# Autodesk Inventor assembly: board_box
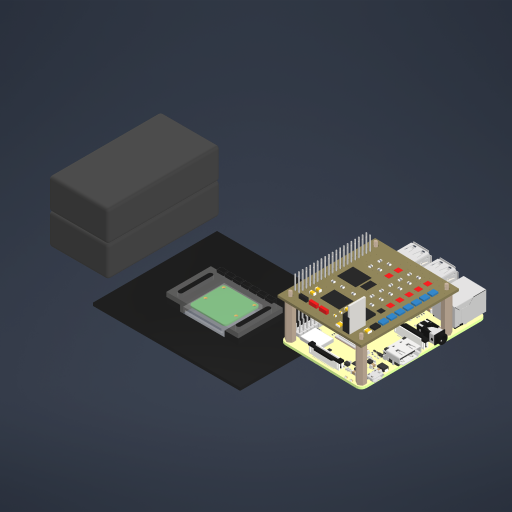
[picture p0: Inventor's stored thumbnail of the model, 512x512]
Saved by Autodesk Inventor 2023 (Build 270158030, 158C)
## iProperties
Created: 2022-07-10
Part Number: board_box
Document SubType Name: Assembly
Designer: Norbert Ligas
Author: Norbert Ligas
## Documents named in this file (8)
- C:\Users\norbe\Repozytoria\NormalMapScanner\3D_modeling\construction\parts\board_box.iam
- C:\Users\norbe\Repozytoria\NormalMapScanner\3D_modeling\power_supply_pcb\power_supply.iam
- C:\Users\norbe\Repozytoria\NormalMapScanner\3D_modeling\construction\spacer23.5_4.5bolt.ipt
- C:\Users\norbe\Repozytoria\NormalMapScanner\3D_modeling\construction\parts\external_parts\raspberry_pi_3_b_plus\raspberry_pi_3_b_plus.iam
- C:\Users\norbe\Repozytoria\NormalMapScanner\3D_modeling\construction\parts\board_box\RaspberryCameraV2InCase.iam
- C:\Users\norbe\Repozytoria\NormalMapScanner\3D_modeling\construction\parts\board_box\board_box_bottom.ipt
- C:\Users\norbe\Repozytoria\NormalMapScanner\3D_modeling\construction\parts\board_box\RaspberryCameraV2Case.ipt
- C:\Users\norbe\Repozytoria\NormalMapScanner\3D_modeling\construction\parts\board_box\accumulators_case.ipt
## Components (10 placed, 6 different names)
1. raspberry_pi_3_b_plus:2 [sub-assembly] — Mate:19, Mate:20, Mate:21, Mate:22, Mate:25
2. power_supply:1 [sub-assembly] — Mate:23, Mate:24, Mate:26
3. spacer23.5_4.5bolt:1 — Mate:20
4. spacer23.5_4.5bolt:2 — Mate:19, Mate:23, Mate:25, Mate:26
5. spacer23.5_4.5bolt:3 — Mate:22
6. spacer23.5_4.5bolt:4 — Mate:21, Mate:24
7. RaspberryCameraV2InCase:1 [sub-assembly] — Mate:27, Flush:1, Flush:2, Mate:29, Mate:30, Mate:31, Mate:32
8. board_box_bottom:1 — Mate:29, Mate:30, Mate:31, Mate:32
9. accumulators_case:1 — Mate:28, Flush:3, Flush:4
10. accumulators_case:2 — Mate:28, Flush:3, Flush:4
## Relationships (18: Mate 14, Flush 4)
- Mate:19: raspberry_pi_3_b_plus:2 ↔ spacer23.5_4.5bolt:2
- Mate:20: raspberry_pi_3_b_plus:2 ↔ spacer23.5_4.5bolt:1
- Mate:21: raspberry_pi_3_b_plus:2 ↔ spacer23.5_4.5bolt:4
- Mate:22: raspberry_pi_3_b_plus:2 ↔ spacer23.5_4.5bolt:3
- Mate:23: power_supply:1 ↔ spacer23.5_4.5bolt:2
- Mate:24: power_supply:1 ↔ spacer23.5_4.5bolt:4
- Mate:25: raspberry_pi_3_b_plus:2 ↔ spacer23.5_4.5bolt:2
- Mate:26: power_supply:1 ↔ spacer23.5_4.5bolt:2
- Mate:27: RaspberryCameraV2InCase:1
- Flush:1: RaspberryCameraV2InCase:1
- Flush:2: RaspberryCameraV2InCase:1
- Mate:28: accumulators_case:1 ↔ accumulators_case:2
- Flush:3: accumulators_case:1 ↔ accumulators_case:2
- Flush:4: accumulators_case:1 ↔ accumulators_case:2
- Mate:29: RaspberryCameraV2InCase:1 ↔ board_box_bottom:1
- Mate:30: RaspberryCameraV2InCase:1 ↔ board_box_bottom:1
- Mate:31: RaspberryCameraV2InCase:1 ↔ board_box_bottom:1
- Mate:32: RaspberryCameraV2InCase:1 ↔ board_box_bottom:1
## Named parameters: bottom_rasp_holder_radius_difference = 1 mm, width = 30.5 mm, length = 49.3 mm, opening_width = 3 mm, opening_length = 23.2 mm, opening_distance_to_edge = 3.3 mm, camera_box_width = 30.5 mm, thickness = 3 mm, inside_width = 26.2 mm, height = 12.3 mm, raspberry_pcb_length = 1 mm, raspberry_pcb_width = 1 mm, power_supply_width = 57.8 mm, power_supply_length = 66.4 mm, board_box_inside_width = 1 mm, board_box_inside_length = 1 mm, batteries_case_width = 41 mm, batteries_case_length = 77 mm, batteries_case_height = 21 mm
